# Autodesk Inventor assembly: CubiertaUnion
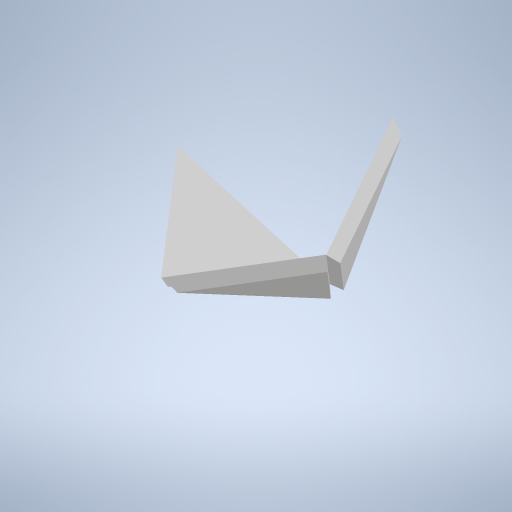
[picture p0: Inventor's stored thumbnail of the model, 512x512]
Saved by Autodesk Inventor 2024 (Build 280153000, 153)
## iProperties
Created: 2024-04-21
Part Number: CubiertaUnion
Document SubType Name: Assembly
Designer: sergi
Author: sergi
## Documents named in this file (2)
- C:\Users\sergi\OneDrive\Escritorio\proyectos\Objetos 3d\pantalla\CubiertaUnion.iam
- C:\Users\sergi\OneDrive\Escritorio\proyectos\Piso\Dodecaedro\Union.ipt
## Components (3 placed, 1 different names)
1. Union:1 — Coincidencia:1, Ángulo:1
2. Union:2 — Coincidencia:1, Ángulo:1, Coincidencia:2, Ángulo:2
3. Union:3 — Coincidencia:2, Ángulo:2
## Relationships (4: Mate 2, Angle 2)
- Coincidencia:1 [Mate]: Union:1 ↔ Union:2
- Ángulo:1 [Angle] (63 deg): Union:1 ↔ Union:2
- Coincidencia:2 [Mate]: Union:2 ↔ Union:3
- Ángulo:2 [Angle] (63 deg): Union:2 ↔ Union:3
